# Autodesk Inventor assembly: atmega
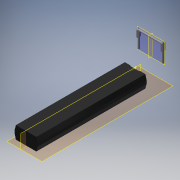
[picture p0: Inventor's stored thumbnail of the model, 180x180]
Saved by Autodesk Inventor 2018 (Build 220112000, 112)
## iProperties
Created: 2017-04-13
Part Number: atmega
Document SubType Name: Assembly
Designer: kampe_000
Author: kampe_000
## Documents named in this file (3)
- D:\Kod\stepCounter\CAD\Inventor Project\assembly\atmega.iam
- D:\Kod\stepCounter\CAD\Inventor Project\parts\atmega_mold.ipt
- D:\Kod\stepCounter\CAD\Inventor Project\parts\atmega_pin.ipt
## Components (2 placed, 2 different names)
1. atmega_mold:1 — Mate:1
2. atmega_pin:1
## Relationships (1: Mate 1)
- Mate:1: atmega_mold:1
## Named parameters: atmegaPinDistance = 2.54 mm
